# Autodesk Inventor assembly: 头部
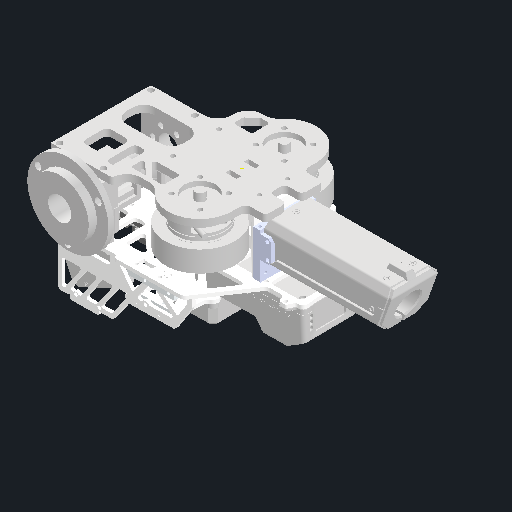
[picture p0: Inventor's stored thumbnail of the model, 512x512]
Saved by Autodesk Inventor 2025 (Build 290162000, 162)
## iProperties
Created: 2024-12-26
Part Number: 头部
Document SubType Name: Assembly
Designer: HZD
Author: HZD
## Documents named in this file (22)
- C:\1A_Engineering_files\GCG全向轮步兵\云台\头部.iam
- C:\1A_Engineering_files\GCG全向轮步兵\云台\零件76.ipt
- C:\1A_Engineering_files\GCG全向轮步兵\云台\零件76_MIR.ipt
- C:\1A_Engineering_files\GCG全向轮步兵\云台\零件152.ipt
- C:\1A_Engineering_files\GCG全向轮步兵\云台\零件79.ipt
- C:\1A_Engineering_files\GCG全向轮步兵\云台\零件80.ipt
- C:\1A_Engineering_files\GCG全向轮步兵\云台\部件9.iam
- C:\1A_Engineering_files\GCG全向轮步兵\云台\零件84.ipt
- C:\1A_Engineering_files\GCG全向轮步兵\云台\零件152_CPY.ipt
- C:\1A_Engineering_files\GCG全向轮步兵\云台\枪管上板1.ipt
- C:\1A_Engineering_files\GCG全向轮步兵\云台\零件85.ipt
- C:\1A_Engineering_files\GCG全向轮步兵\云台\发射机构侧板.ipt
- C:\1A_Engineering_files\GCG全向轮步兵\云台\吊装色相头.ipt
- C:\1A_Engineering_files\GCG全向轮步兵\云台\发射机构侧板1.ipt
- C:\1A_Engineering_files\GCG全向轮步兵\云台\枪管固定加工件-v1.0.ipt
- C:\1A_Engineering_files\GCG全向轮步兵\云台\M3四孔长连接件.ipt
- C:\1A_Engineering_files\GCG全向轮步兵\云台\C620无刷电机调速器.ipt
- C:\1A_Engineering_files\GCG全向轮步兵\云台\a板摆放.iam
- C:\1A_Engineering_files\GCG全向轮步兵\云台\陀螺仪1.ipt
- C:\1A_Engineering_files\GCG哨兵\云台\云台装配体\充能\3D_LEDboard_2024-10-09_MIR.ipt
- C:\1A_Engineering_files\GCG全向轮步兵\云台\4mm隔热板.ipt
- C:\1A_Engineering_files\GCG全向轮步兵\云台\枪管座(2).ipt
## Components (24 placed, 21 different names)
1. 零件76:1 — 配合:54, 配合:75, 配合:76, 配合:81, 配合:82
2. 零件76_MIR:1 — 配合:55
3. 零件79:1 — 配合:52, 配合:53, 配合:54
4. 零件80:1 — 配合:16, 配合:17, 配合:18, 配合:19, 配合:22, 配合:51, 配合:56, 配合:59
5. 部件9:1 [sub-assembly] — 配合:16, 配合:17
6. 部件9:2 [sub-assembly] — 配合:18, 配合:19
7. 零件84:1 — 配合:44
8. 零件152_CPY:1 — 配合:22, 配合:56, 配合:57, 配合:60
9. 枪管上板1:1 — 配合:24, 配合:25, 配合:26, 配合:27, 配合:34, 配合:35, 配合:39, 配合:40, 配合:41, 配合:57, 配合:58, 配合:60, 配合:63, 配合:64, 配合:72, 配合:73, 配合:74
10. 零件85:1 — 配合:24, 配合:25, 配合:26, 配合:27
11. 发射机构侧板:2 — 配合:34, 配合:35, 配合:37, 配合:38, 配合:42, 配合:47, 配合:67, 配合:69, 配合:70, 表面齐平:2
12. 吊装色相头:1 — 配合:37, 配合:38, 配合:42, 配合:77, 表面齐平:1
13. 发射机构侧板1:1 — 配合:39, 配合:40, 配合:41, 配合:65, 表面齐平:2
14. 枪管固定加工件-v1.0:1 — 配合:44, 配合:78, 配合:79, 配合:80
15. M3四孔长连接件:1 — 配合:47, 配合:63, 配合:64
16. 零件152:2 — 配合:51, 配合:52, 配合:53, 配合:55, 配合:58, 配合:59
17. C620无刷电机调速器:1 — 配合:65, 配合:68, 配合:71
18. C620无刷电机调速器:2 — 配合:67, 配合:68, 配合:71
19. M3四孔长连接件:2 — 配合:69, 配合:70
20. a板摆放:1 [sub-assembly] — 配合:72, 配合:73, 配合:74
21. 陀螺仪1:1 — 配合:77, 表面齐平:1
22. 3D_LEDboard_2024-10-09_MIR:1
23. 4mm隔热板:1 — 配合:75, 配合:76
24. 枪管座(2):1 — 配合:78, 配合:79, 配合:80, 配合:81, 配合:82
## Relationships (50: Mate 48, Flush 2)
- 配合:16 [Mate]: 零件80:1 ↔ 部件9:1
- 配合:17 [Mate]: 零件80:1 ↔ 部件9:1
- 配合:18 [Mate]: 零件80:1 ↔ 部件9:2
- 配合:19 [Mate]: 零件80:1 ↔ 部件9:2
- 配合:22 [Mate]: 零件80:1 ↔ 零件152_CPY:1
- 配合:24 [Mate]: 枪管上板1:1 ↔ 零件85:1
- 配合:25 [Mate]: 枪管上板1:1 ↔ 零件85:1
- 配合:26 [Mate]: 枪管上板1:1 ↔ 零件85:1
- 配合:27 [Mate]: 枪管上板1:1 ↔ 零件85:1
- 配合:34 [Mate]: 枪管上板1:1 ↔ 发射机构侧板:2
- 配合:35 [Mate]: 枪管上板1:1 ↔ 发射机构侧板:2
- 配合:37 [Mate]: 发射机构侧板:2 ↔ 吊装色相头:1
- 配合:38 [Mate]: 发射机构侧板:2 ↔ 吊装色相头:1
- 配合:39 [Mate]: 枪管上板1:1 ↔ 发射机构侧板1:1
- 配合:40 [Mate]: 枪管上板1:1 ↔ 发射机构侧板1:1
- 配合:41 [Mate]: 枪管上板1:1 ↔ 发射机构侧板1:1
- 配合:42 [Mate]: 发射机构侧板:2 ↔ 吊装色相头:1
- 配合:44 [Mate]: 零件84:1 ↔ 枪管固定加工件-v1.0:1
- 配合:47 [Mate]: 发射机构侧板:2 ↔ M3四孔长连接件:1
- 配合:51 [Mate]: 零件80:1 ↔ 零件152:2
- 配合:52 [Mate]: 零件79:1 ↔ 零件152:2
- 配合:53 [Mate]: 零件79:1 ↔ 零件152:2
- 配合:54 [Mate]: 零件76:1 ↔ 零件79:1
- 配合:55 [Mate]: 零件76_MIR:1 ↔ 零件152:2
- 配合:56 [Mate]: 零件80:1 ↔ 零件152_CPY:1
- 配合:57 [Mate]: 零件152_CPY:1 ↔ 枪管上板1:1
- 配合:58 [Mate]: 枪管上板1:1 ↔ 零件152:2
- 配合:59 [Mate]: 零件80:1 ↔ 零件152:2
- 配合:60 [Mate]: 零件152_CPY:1 ↔ 枪管上板1:1
- 配合:63 [Mate]: 枪管上板1:1 ↔ M3四孔长连接件:1
- 配合:64 [Mate]: 枪管上板1:1 ↔ M3四孔长连接件:1
- 配合:65 [Mate]: 发射机构侧板1:1 ↔ C620无刷电机调速器:1
- 配合:67 [Mate]: 发射机构侧板:2 ↔ C620无刷电机调速器:2
- 配合:68 [Mate]: C620无刷电机调速器:1 ↔ C620无刷电机调速器:2
- 配合:69 [Mate]: 发射机构侧板:2 ↔ M3四孔长连接件:2
- 配合:70 [Mate]: 发射机构侧板:2 ↔ M3四孔长连接件:2
- 配合:71 [Mate]: C620无刷电机调速器:1 ↔ C620无刷电机调速器:2
- 配合:72 [Mate]: 枪管上板1:1 ↔ a板摆放:1
- 配合:73 [Mate]: 枪管上板1:1 ↔ a板摆放:1
- 配合:74 [Mate]: 枪管上板1:1 ↔ a板摆放:1
- 配合:75 [Mate]: 零件76:1 ↔ 4mm隔热板:1
- 配合:76 [Mate]: 零件76:1 ↔ 4mm隔热板:1
- 配合:77 [Mate]: 吊装色相头:1 ↔ 陀螺仪1:1
- 表面齐平:1 [Flush]: 吊装色相头:1 ↔ 陀螺仪1:1
- 表面齐平:2 [Flush]: 发射机构侧板:2 ↔ 发射机构侧板1:1
- 配合:78 [Mate]: 枪管固定加工件-v1.0:1 ↔ 枪管座(2):1
- 配合:79 [Mate]: 枪管固定加工件-v1.0:1 ↔ 枪管座(2):1
- 配合:80 [Mate]: 枪管固定加工件-v1.0:1 ↔ 枪管座(2):1
- 配合:81 [Mate]: 零件76:1 ↔ 枪管座(2):1
- 配合:82 [Mate]: 零件76:1 ↔ 枪管座(2):1
